# Autodesk Inventor assembly: Carcasa_Soldada
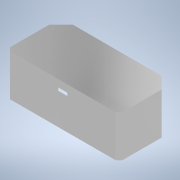
[picture p0: Inventor's stored thumbnail of the model, 180x180]
Saved by Autodesk Inventor 2022.1 (Build 261234000, 234)
## iProperties
Created: 2021-10-29
Part Number: Carcasa_Soldada
Document SubType Name: Weldment
Designer: seb_0
Weld Material: Welded Aluminum-6061
Author: seb_0
## Documents named in this file (3)
- C:\Users\seb_0\Desktop\PDM\ProyectoRobotPallet\Carcasa\Carcasa_Soldada.iam
- C:\Users\seb_0\Desktop\PDM\ProyectoRobotPallet\Carcasa\Carcasa.ipt
- C:\Users\seb_0\Desktop\PDM\ProyectoRobotPallet\Carcasa\Cubo.ipt
## Components (7 placed, 2 different names)
1. Carcasa:1 — Coincidencia:1, Coincidencia:2, Coincidencia:3, Coincidencia:4, Nivelación:1, Nivelación:2, Coincidencia:5, Coincidencia:6, Nivelación:4, Nivelación:5, Coincidencia:7, Coincidencia:8, Nivelación:7, Nivelación:8
2. Cubo:1 — Coincidencia:6, Nivelación:5, Nivelación:6
3. Cubo:2 — Coincidencia:5, Nivelación:4, Nivelación:6
4. Cubo:3 — Coincidencia:8, Nivelación:8, Nivelación:9
5. Cubo:4 — Coincidencia:7, Nivelación:7, Nivelación:9
6. Cubo:5 — Coincidencia:3, Nivelación:1, Nivelación:3
7. Cubo:6 — Coincidencia:4, Nivelación:2, Nivelación:3
## Relationships (17: Flush 9, Mate 8)
- Coincidencia:1 [Mate]: Carcasa:1
- Coincidencia:2 [Mate]: Carcasa:1
- Coincidencia:3 [Mate]: Carcasa:1 ↔ Cubo:5
- Coincidencia:4 [Mate]: Carcasa:1 ↔ Cubo:6
- Nivelación:1 [Flush] (15 mm): Carcasa:1 ↔ Cubo:5
- Nivelación:2 [Flush] (15 mm): Carcasa:1 ↔ Cubo:6
- Nivelación:3 [Flush]: Cubo:5 ↔ Cubo:6
- Coincidencia:5 [Mate]: Carcasa:1 ↔ Cubo:2
- Coincidencia:6 [Mate]: Carcasa:1 ↔ Cubo:1
- Nivelación:4 [Flush] (15 mm): Carcasa:1 ↔ Cubo:2
- Nivelación:5 [Flush] (15 mm): Carcasa:1 ↔ Cubo:1
- Nivelación:6 [Flush]: Cubo:1 ↔ Cubo:2
- Coincidencia:7 [Mate]: Carcasa:1 ↔ Cubo:4
- Coincidencia:8 [Mate]: Carcasa:1 ↔ Cubo:3
- Nivelación:7 [Flush] (15 mm): Carcasa:1 ↔ Cubo:4
- Nivelación:8 [Flush] (15 mm): Carcasa:1 ↔ Cubo:3
- Nivelación:9 [Flush]: Cubo:3 ↔ Cubo:4
